# Autodesk Inventor assembly: 000200
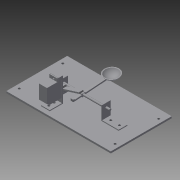
[picture p0: Inventor's stored thumbnail of the model, 180x180]
Saved by Autodesk Inventor 2015 (Build 190159000, 159)
## iProperties
Created: 2015-05-29
Part Number: 000200
Document SubType Name: Assembly
Designer: Wesley
Author: Wesley
## Documents named in this file (8)
- C:\Users\Wesley\Documents\GitHub\EngineeringFinal\Engineering\Engineering Documentation\CADS\0002__\000200.iam
- C:\Users\Wesley\Documents\GitHub\EngineeringFinal\Engineering\Engineering Documentation\CADS\0002__\000201.ipt
- C:\Users\Wesley\Documents\GitHub\EngineeringFinal\Engineering\Engineering Documentation\CADS\0002__\000204.ipt
- C:\Users\Wesley\Documents\GitHub\EngineeringFinal\Engineering\Engineering Documentation\CADS\0002__\000203.ipt
- C:\Users\Wesley\Documents\GitHub\EngineeringFinal\Engineering\Engineering Documentation\CADS\0002__\000205.ipt
- C:\Users\Wesley\Documents\GitHub\EngineeringFinal\Engineering\Engineering Documentation\CADS\0002__\000208.ipt
- C:\Users\Wesley\Documents\GitHub\EngineeringFinal\Engineering\Engineering Documentation\CADS\0002__\000206.ipt
- C:\Users\Wesley\Documents\GitHub\EngineeringFinal\Engineering\Engineering Documentation\CADS\0002__\000207.ipt
## Components (8 placed, 7 different names)
1. 000201:1 — Mate:1, Mate:2, Mate:3, Mate:4, Mate:5, Mate:6, Mate:7, Mate:8, Mate:9, Mate:13, Mate:14, Mate:15
2. 000204:1 — Mate:4, Mate:5, Mate:6
3. 000204:2 — Mate:7, Mate:8, Mate:9, Mate:10, Mate:12
4. 000203:1 — Mate:10, Mate:11
5. 000205:1 — Mate:11, Mate:12
6. 000208:1 — Mate:13, Mate:14, Mate:15, Mate:16, Mate:17, Mate:19
7. 000206:1 — Mate:16, Mate:17, Mate:18, Mate:19, Mate:20
8. 000207:1 — Mate:18, Mate:20
## Relationships (20: Mate 20)
- Mate:1: 000201:1
- Mate:2: 000201:1
- Mate:3: 000201:1
- Mate:4: 000201:1 ↔ 000204:1
- Mate:5: 000201:1 ↔ 000204:1
- Mate:6: 000201:1 ↔ 000204:1
- Mate:7: 000201:1 ↔ 000204:2
- Mate:8: 000201:1 ↔ 000204:2
- Mate:9: 000201:1 ↔ 000204:2
- Mate:10: 000204:2 ↔ 000203:1
- Mate:11: 000203:1 ↔ 000205:1
- Mate:12 (31.75 mm): 000204:2 ↔ 000205:1
- Mate:13: 000201:1 ↔ 000208:1
- Mate:14: 000201:1 ↔ 000208:1
- Mate:15: 000201:1 ↔ 000208:1
- Mate:16: 000208:1 ↔ 000206:1
- Mate:17: 000208:1 ↔ 000206:1
- Mate:18: 000206:1 ↔ 000207:1
- Mate:19: 000208:1 ↔ 000206:1
- Mate:20 (0.254 mm): 000206:1 ↔ 000207:1
